# Autodesk Inventor assembly: XaxisAssem
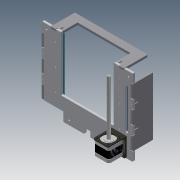
[picture p0: Inventor's stored thumbnail of the model, 180x180]
Saved by Autodesk Inventor 2014 (Build 180170000, 170)
## iProperties
Created: 2015-01-19
Part Number: XaxisAssem
Document SubType Name: Assembly
Designer: Peele
Author: Peele
## Documents named in this file (7)
- E:\Copy\DLP\PandaPrint\CustomParts\XaxisAssem.iam
- E:\Copy\DLP\PandaPrint\CustomParts\InnerTop.ipt
- E:\Copy\DLP\PandaPrint\StockParts\Rail.ipt
- E:\Copy\DLP\PandaPrint\StockParts\Rail\Rail-06.ipt
- E:\Copy\DLP\PandaPrint\SubAssem\StepperWithMount.iam
- E:\Copy\DLP\PandaPrint\CustomParts\InnerSide.ipt
- E:\Copy\DLP\PandaPrint\CustomParts\InnerFront.ipt
## Components (7 placed, 5 different names)
1. InnerTop:1 — Mate:1, Mate:2, Flush:1, Mate:3, Flush:6, Mate:4, Flush:7, Tangent:1, Flush:8, Flush:9, Flush:10, Flush:11, Flush:12, Flush:14, Flush:15
2. Rail-06:1 — Mate:3, Flush:2, Flush:3, Flush:5
3. Rail-06:2 — Flush:2, Flush:4, Flush:5, Flush:6
4. StepperWithMount:1 [sub-assembly] — Mate:4, Flush:7, Tangent:1
5. InnerSide:1 — Flush:8, Flush:9, Flush:10, Flush:13
6. InnerSide:2 — Flush:11, Flush:12, Flush:13
7. InnerFront:1 — Flush:14, Flush:15, Mate:5
## Relationships (21: Flush 15, Mate 5, Tangent 1)
- Mate:1: InnerTop:1
- Mate:2: InnerTop:1
- Flush:1: InnerTop:1
- Mate:3: InnerTop:1 ↔ Rail-06:1
- Flush:2: Rail-06:1 ↔ Rail-06:2
- Flush:3 (87.5 mm): Rail-06:1
- Flush:4 (-87.5 mm): Rail-06:2
- Flush:5: Rail-06:1 ↔ Rail-06:2
- Flush:6 (15 mm): InnerTop:1 ↔ Rail-06:2
- Mate:4: InnerTop:1 ↔ StepperWithMount:1
- Flush:7: InnerTop:1 ↔ StepperWithMount:1
- Tangent:1: InnerTop:1 ↔ StepperWithMount:1
- Flush:8: InnerTop:1 ↔ InnerSide:1
- Flush:9 (-25 mm): InnerTop:1 ↔ InnerSide:1
- Flush:10: InnerTop:1 ↔ InnerSide:1
- Flush:11: InnerTop:1 ↔ InnerSide:2
- Flush:12: InnerTop:1 ↔ InnerSide:2
- Flush:13: InnerSide:1 ↔ InnerSide:2
- Flush:14: InnerTop:1 ↔ InnerFront:1
- Flush:15: InnerTop:1 ↔ InnerFront:1
- Mate:5: InnerFront:1
